# Autodesk Inventor assembly: Assembly_microfluidic_chip
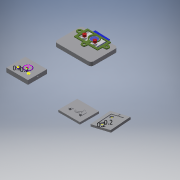
[picture p0: Inventor's stored thumbnail of the model, 180x180]
Saved by Autodesk Inventor 2019.4 (Build 234330000, 330)
## iProperties
Created: 2021-04-19
Part Number: Assembly_microfluidic_chip
Document SubType Name: Assembly
Designer: diederichbenedict
Author: diederichbenedict
## Documents named in this file (9)
- C:\Users\diederichbenedict\Dropbox\Dokumente\Promotion\PROJECTS\STORMoChip\GITHUB\CAD\Nanoscopy-on-the-cheap\Workspace\Assembly_microfluidic_chip.iam
- C:\Users\diederichbenedict\Dropbox\Dokumente\Promotion\PROJECTS\STORMoChip\GITHUB\CAD\Nanoscopy-on-the-cheap\Workspace\cellSTORM_v5_chiptray_brightfieldslide.ipt
- C:\Users\diederichbenedict\Dropbox\Dokumente\Promotion\PROJECTS\STORMoChip\GITHUB\CAD\Nanoscopy-on-the-cheap\Workspace\00_chip_01_new.ipt
- C:\Users\diederichbenedict\Dropbox\Dokumente\Promotion\PROJECTS\STORMoChip\GITHUB\CAD\Nanoscopy-on-the-cheap\Workspace\00_fluidic_input.ipt
- C:\Users\diederichbenedict\Dropbox\Dokumente\Promotion\PROJECTS\STORMoChip\GITHUB\CAD\Nanoscopy-on-the-cheap\Workspace\00_roundcoverslip_12mm.ipt
- C:\Users\diederichbenedict\Dropbox\Dokumente\Promotion\PROJECTS\STORMoChip\GITHUB\CAD\Nanoscopy-on-the-cheap\Workspace\00_PDMS_chamber_fluidic_v0.ipt
- C:\Users\diederichbenedict\Dropbox\Dokumente\Promotion\PROJECTS\STORMoChip\GITHUB\CAD\Nanoscopy-on-the-cheap\Workspace\00_PDMS_chamber_clamp.ipt
- C:\Users\diederichbenedict\Dropbox\Dokumente\Promotion\PROJECTS\STORMoChip\GITHUB\CAD\Nanoscopy-on-the-cheap\Workspace\00_PDMS_mould_0.ipt
- C:\Users\diederichbenedict\Dropbox\Dokumente\Promotion\PROJECTS\STORMoChip\GITHUB\CAD\Nanoscopy-on-the-cheap\Workspace\00_PDMS_mould_1.ipt
## Components (12 placed, 8 different names)
1. cellSTORM_v5_chiptray_brightfieldslide:1 — Mate:1
2. 00_chip_01_new:1 — Mate:1, Mate:2, Mate:3, Mate:5, Mate:6, Flush:1, Mate:7, Flush:2, Flush:3
3. 00_fluidic_input:1 — Mate:2, Mate:4, Mate:5, Mate:6
4. 00_roundcoverslip_12mm:1 — Mate:3
5. 00_fluidic_input:2 — Mate:4, Flush:1, Mate:7
6. 00_PDMS_chamber_fluidic_v0:1 — Flush:2, Flush:3, Flush:4, Flush:5
7. 00_PDMS_chamber_clamp:1 — Flush:4, Flush:5
8. 00_PDMS_chamber_fluidic_v0:2 — Flush:6, Flush:7
9. 00_PDMS_mould_0:1 — Flush:6, Flush:7, Flush:8, Flush:9
10. 00_PDMS_mould_1:1 — Flush:8, Flush:9
11. 00_PDMS_mould_1:2
12. 00_PDMS_mould_0:2
## Relationships (16: Flush 9, Mate 7)
- Mate:1: cellSTORM_v5_chiptray_brightfieldslide:1 ↔ 00_chip_01_new:1
- Mate:2 (1 mm): 00_chip_01_new:1 ↔ 00_fluidic_input:1
- Mate:3 (0.6 mm): 00_chip_01_new:1 ↔ 00_roundcoverslip_12mm:1
- Mate:4: 00_fluidic_input:1 ↔ 00_fluidic_input:2
- Mate:5 (-3.5 mm): 00_chip_01_new:1 ↔ 00_fluidic_input:1
- Mate:6 (-3.5 mm): 00_chip_01_new:1 ↔ 00_fluidic_input:1
- Flush:1 (3.5 mm): 00_chip_01_new:1 ↔ 00_fluidic_input:2
- Mate:7 (-3.5 mm): 00_chip_01_new:1 ↔ 00_fluidic_input:2
- Flush:2: 00_chip_01_new:1 ↔ 00_PDMS_chamber_fluidic_v0:1
- Flush:3: 00_chip_01_new:1 ↔ 00_PDMS_chamber_fluidic_v0:1
- Flush:4: 00_PDMS_chamber_fluidic_v0:1 ↔ 00_PDMS_chamber_clamp:1
- Flush:5: 00_PDMS_chamber_fluidic_v0:1 ↔ 00_PDMS_chamber_clamp:1
- Flush:6: 00_PDMS_chamber_fluidic_v0:2 ↔ 00_PDMS_mould_0:1
- Flush:7: 00_PDMS_chamber_fluidic_v0:2 ↔ 00_PDMS_mould_0:1
- Flush:8: 00_PDMS_mould_0:1 ↔ 00_PDMS_mould_1:1
- Flush:9: 00_PDMS_mould_0:1 ↔ 00_PDMS_mould_1:1
